# Autodesk Inventor assembly: assembly
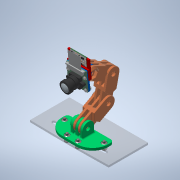
[picture p0: Inventor's stored thumbnail of the model, 180x180]
Saved by Autodesk Inventor 2020 (Build 240168000, 168)
## iProperties
Created: 2019-10-09
Part Number: assembly
Document SubType Name: Assembly
Designer: ZEUSLAP
Author: ZEUSLAP
## Documents named in this file (15)
- C:\data\Tonic\cad\camera_mount\assembly_imu.iam
- C:\data\Tonic\cad\camera_mount\platform_parts\platform.ipt
- C:\data\Tonic\cad\camera_mount\printable\camera_mount.ipt
- C:\data\Tonic\cad\camera_mount\printable\platform_mount.ipt
- C:\data\Tonic\cad\camera_mount\platform_parts\camera\Raspberry Pi Camera (G) 160 deg.iam
- C:\data\Tonic\cad\camera_mount\printable\arm-30-straight-v5-1.ipt
- C:\Users\Vadim\Documents\Inventor\Content Center Files\R2020\en-US\ISO 4035(2)\ISO 4035 - M3 - ISO.ipt
- C:\Users\Vadim\Documents\Inventor\Content Center Files\R2020\en-US\SFS EN ISO 7045 Z\EN ISO 7045 - M3 x 8 - 4.8 - Z(3).ipt
- C:\Users\Vadim\Documents\Inventor\Content Center Files\R2020\en-US\SFS EN ISO 7045 Z\EN ISO 7045 - M2 x 5 - 4.8 - Z(3).ipt
- C:\Users\Vadim\Documents\Inventor\Content Center Files\R2020\en-US\ISO 4035(2)\ISO 4035 - M2 - ISO.ipt
- C:\data\Tonic\cad\camera_mount\printable\imu_mount.ipt
- C:\data\Tonic\cad\camera_mount\platform_parts\minimu-9.ipt
- C:\Users\Vadim\Documents\Inventor\Content Center Files\R2020\en-US\SFS EN ISO 7045 Z\EN ISO 7045 - M2 x 4 - 4.8 - Z(3).ipt
- C:\Users\Vadim\Documents\Inventor\Content Center Files\R2020\en-US\SFS EN ISO 7045 Z\EN ISO 7045 - M2 x 8 - 4.8 - Z(3).ipt
- C:\Users\Vadim\Documents\Inventor\Content Center Files\R2020\en-US\SFS EN ISO 7045 Z\EN ISO 7045 - M1.6 x 3 - 4.8 - Z(3).ipt
## Components (29 placed, 14 different names)
1. platform:1 — Mate:1, Mate:2, Mate:3, Mate:46, Mate:47, Mate:48, Mate:49, Mate:50, Mate:51, Mate:52, Mate:53, Mate:65, Mate:66
2. camera_mount:1 — Mate:10, Mate:11, Mate:12, Mate:13, Mate:41, Mate:45, Mate:62, Mate:63, Mate:64
3. platform_mount:1 — Mate:1, Mate:2, Mate:3, Mate:4, Mate:5, Mate:55, Mate:57, Mate:59, Mate:61, Angle:1, Angle:2, Angle:3, Angle:4
4. Raspberry Pi Camera (G) 160 deg:1 [sub-assembly] — Mate:12, Mate:13, Mate:34, Mate:35, Mate:36, Mate:37, Mate:78, Mate:79, Mate:82, Mate:83, Mate:85, Mate:87
5. arm-30-straight-v5-1:1 — Mate:8, Mate:9, Mate:10, Mate:11
6. arm-30-straight-v5-1:2 — Mate:4, Mate:5, Mate:6, Mate:7
7. arm-30-straight-v5-1:3 — Mate:6, Mate:7, Mate:8, Mate:9
8. SFS EN ISO 7045 Z M2 x 5 - 4.8 - Z:3 — Mate:34, Mate:35, Mate:44
9. SFS EN ISO 7045 Z M2 x 5 - 4.8 - Z:4 — Mate:36, Mate:37, Mate:40
10. ISO 4035 M2:2 — Mate:40, Mate:41
11. ISO 4035 M2:4 — Mate:44, Mate:45
12. SFS EN ISO 7045 Z M3 x 8 - 4.8 - Z:1 — Mate:46, Mate:47, Mate:56
13. SFS EN ISO 7045 Z M3 x 8 - 4.8 - Z:2 — Mate:48, Mate:49, Mate:58
14. SFS EN ISO 7045 Z M3 x 8 - 4.8 - Z:3 — Mate:50, Mate:51, Mate:54
15. SFS EN ISO 7045 Z M3 x 8 - 4.8 - Z:4 — Mate:52, Mate:53, Mate:60
16. ISO 4035 M3:1 — Mate:54, Mate:55, Angle:2
17. ISO 4035 M3:2 — Mate:56, Mate:57, Angle:3
18. ISO 4035 M3:3 — Mate:58, Mate:59, Angle:4
19. ISO 4035 M3:4 — Mate:60, Mate:61, Angle:1
20. imu_mount:1 — Mate:62, Mate:63, Mate:64, Mate:68, Mate:69, Mate:75, Mate:84, Mate:86, Angle:5, Mate:91, Mate:92
21. minimu-9:1 — Mate:68, Mate:69, Mate:72, Mate:73, Angle:5
22. SFS EN ISO 7045 Z M2 x 4 - 4.8 - Z:1 — Mate:72, Mate:73, Mate:74
23. ISO 4035 M2:5 — Mate:74, Mate:75
24. SFS EN ISO 7045 Z M1.6 x 3 - 4.8 - Z:2 — Mate:78, Mate:79
25. SFS EN ISO 7045 Z M1.6 x 3 - 4.8 - Z:4 — Mate:82, Mate:83
26. SFS EN ISO 7045 Z M2 x 8 - 4.8 - Z:1 — Mate:84, Mate:85, Mate:88
27. SFS EN ISO 7045 Z M2 x 8 - 4.8 - Z:2 — Mate:86, Mate:87, Mate:90
28. ISO 4035 M2:6 — Mate:88, Mate:91
29. ISO 4035 M2:7 — Mate:90, Mate:92
## Relationships (65: Mate 60, Angle 5)
- Mate:1: platform:1 ↔ platform_mount:1
- Mate:2: platform:1 ↔ platform_mount:1
- Mate:3: platform:1 ↔ platform_mount:1
- Mate:4: platform_mount:1 ↔ arm-30-straight-v5-1:2
- Mate:5: platform_mount:1 ↔ arm-30-straight-v5-1:2
- Mate:6: arm-30-straight-v5-1:2 ↔ arm-30-straight-v5-1:3
- Mate:7: arm-30-straight-v5-1:2 ↔ arm-30-straight-v5-1:3
- Mate:8: arm-30-straight-v5-1:1 ↔ arm-30-straight-v5-1:3
- Mate:9: arm-30-straight-v5-1:1 ↔ arm-30-straight-v5-1:3
- Mate:10: camera_mount:1 ↔ arm-30-straight-v5-1:1
- Mate:11: camera_mount:1 ↔ arm-30-straight-v5-1:1
- Mate:12: camera_mount:1 ↔ Raspberry Pi Camera (G) 160 deg:1
- Mate:13: camera_mount:1 ↔ Raspberry Pi Camera (G) 160 deg:1
- Mate:34: Raspberry Pi Camera (G) 160 deg:1 ↔ SFS EN ISO 7045 Z M2 x 5 - 4.8 - Z:3
- Mate:35: Raspberry Pi Camera (G) 160 deg:1 ↔ SFS EN ISO 7045 Z M2 x 5 - 4.8 - Z:3
- Mate:36: Raspberry Pi Camera (G) 160 deg:1 ↔ SFS EN ISO 7045 Z M2 x 5 - 4.8 - Z:4
- Mate:37: Raspberry Pi Camera (G) 160 deg:1 ↔ SFS EN ISO 7045 Z M2 x 5 - 4.8 - Z:4
- Mate:40: SFS EN ISO 7045 Z M2 x 5 - 4.8 - Z:4 ↔ ISO 4035 M2:2
- Mate:41: camera_mount:1 ↔ ISO 4035 M2:2
- Mate:44: SFS EN ISO 7045 Z M2 x 5 - 4.8 - Z:3 ↔ ISO 4035 M2:4
- Mate:45: camera_mount:1 ↔ ISO 4035 M2:4
- Mate:46: platform:1 ↔ SFS EN ISO 7045 Z M3 x 8 - 4.8 - Z:1
- Mate:47: platform:1 ↔ SFS EN ISO 7045 Z M3 x 8 - 4.8 - Z:1
- Mate:48: platform:1 ↔ SFS EN ISO 7045 Z M3 x 8 - 4.8 - Z:2
- Mate:49: platform:1 ↔ SFS EN ISO 7045 Z M3 x 8 - 4.8 - Z:2
- Mate:50: platform:1 ↔ SFS EN ISO 7045 Z M3 x 8 - 4.8 - Z:3
- Mate:51: platform:1 ↔ SFS EN ISO 7045 Z M3 x 8 - 4.8 - Z:3
- Mate:52: platform:1 ↔ SFS EN ISO 7045 Z M3 x 8 - 4.8 - Z:4
- Mate:53: platform:1 ↔ SFS EN ISO 7045 Z M3 x 8 - 4.8 - Z:4
- Mate:54: SFS EN ISO 7045 Z M3 x 8 - 4.8 - Z:3 ↔ ISO 4035 M3:1
- Mate:55: platform_mount:1 ↔ ISO 4035 M3:1
- Mate:56: SFS EN ISO 7045 Z M3 x 8 - 4.8 - Z:1 ↔ ISO 4035 M3:2
- Mate:57: platform_mount:1 ↔ ISO 4035 M3:2
- Mate:58: SFS EN ISO 7045 Z M3 x 8 - 4.8 - Z:2 ↔ ISO 4035 M3:3
- Mate:59: platform_mount:1 ↔ ISO 4035 M3:3
- Mate:60: SFS EN ISO 7045 Z M3 x 8 - 4.8 - Z:4 ↔ ISO 4035 M3:4
- Mate:61: platform_mount:1 ↔ ISO 4035 M3:4
- Angle:1 (90 deg): platform_mount:1 ↔ ISO 4035 M3:4
- Angle:2 (90 deg): platform_mount:1 ↔ ISO 4035 M3:1
- Angle:3 (90 deg): platform_mount:1 ↔ ISO 4035 M3:2
- Angle:4 (90 deg): platform_mount:1 ↔ ISO 4035 M3:3
- Mate:62: camera_mount:1 ↔ imu_mount:1
- Mate:63: camera_mount:1 ↔ imu_mount:1
- Mate:64: camera_mount:1 ↔ imu_mount:1
- Mate:65: platform:1
- Mate:66: platform:1
- Mate:68: imu_mount:1 ↔ minimu-9:1
- Mate:69: imu_mount:1 ↔ minimu-9:1
- Mate:72: minimu-9:1 ↔ SFS EN ISO 7045 Z M2 x 4 - 4.8 - Z:1
- Mate:73: minimu-9:1 ↔ SFS EN ISO 7045 Z M2 x 4 - 4.8 - Z:1
- Mate:74: SFS EN ISO 7045 Z M2 x 4 - 4.8 - Z:1 ↔ ISO 4035 M2:5
- Mate:75: imu_mount:1 ↔ ISO 4035 M2:5
- Mate:78: Raspberry Pi Camera (G) 160 deg:1 ↔ SFS EN ISO 7045 Z M1.6 x 3 - 4.8 - Z:2
- Mate:79: Raspberry Pi Camera (G) 160 deg:1 ↔ SFS EN ISO 7045 Z M1.6 x 3 - 4.8 - Z:2
- Mate:82: Raspberry Pi Camera (G) 160 deg:1 ↔ SFS EN ISO 7045 Z M1.6 x 3 - 4.8 - Z:4
- Mate:83: Raspberry Pi Camera (G) 160 deg:1 ↔ SFS EN ISO 7045 Z M1.6 x 3 - 4.8 - Z:4
- Mate:84: imu_mount:1 ↔ SFS EN ISO 7045 Z M2 x 8 - 4.8 - Z:1
- Mate:85: Raspberry Pi Camera (G) 160 deg:1 ↔ SFS EN ISO 7045 Z M2 x 8 - 4.8 - Z:1
- Mate:86: imu_mount:1 ↔ SFS EN ISO 7045 Z M2 x 8 - 4.8 - Z:2
- Mate:87: Raspberry Pi Camera (G) 160 deg:1 ↔ SFS EN ISO 7045 Z M2 x 8 - 4.8 - Z:2
- Mate:88: SFS EN ISO 7045 Z M2 x 8 - 4.8 - Z:1 ↔ ISO 4035 M2:6
- Mate:90: SFS EN ISO 7045 Z M2 x 8 - 4.8 - Z:2 ↔ ISO 4035 M2:7
- Angle:5 (270 deg): imu_mount:1 ↔ minimu-9:1
- Mate:91: imu_mount:1 ↔ ISO 4035 M2:6
- Mate:92: imu_mount:1 ↔ ISO 4035 M2:7
